# Autodesk Inventor assembly: Wheel_and_Tire_MIR_MIR
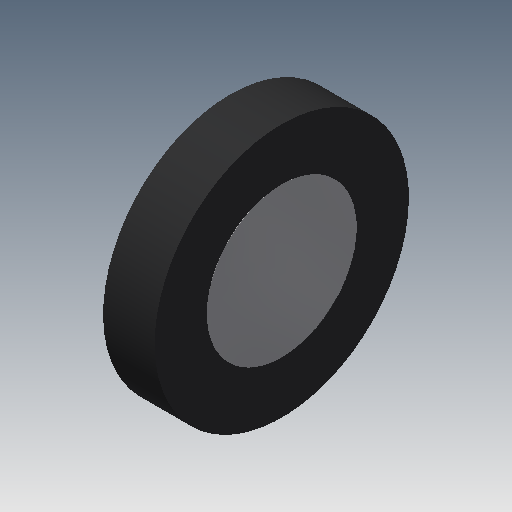
[picture p0: Inventor's stored thumbnail of the model, 512x512]
Saved by Autodesk Inventor 2018 (Build 220112000, 112)
## iProperties
Created: 2017-08-21
Part Number: Wheel_and_Tire_MIR_MIR
Document SubType Name: Assembly
Designer: thoma
Author: thoma
## Documents named in this file (3)
- C:\Users\thoma\Desktop\Tiny_House\Trailer\Wheel_and_Tire_MIR_MIR.iam
- C:\Users\thoma\Desktop\Tiny_House\Trailer\Wheel_MIR_MIR.ipt
- C:\Users\thoma\Desktop\Tiny_House\Trailer\Tire_MIR_MIR.ipt
## Components (2 placed, 2 different names)
1. Wheel_MIR_MIR:1 — Insert:1
2. Tire_MIR_MIR:1 — Insert:1
## Relationships (1: Insert 1)
- Insert:1: Wheel_MIR_MIR:1 ↔ Tire_MIR_MIR:1
